# Autodesk Inventor assembly: Extended 5 frame Hole Top and Bottom
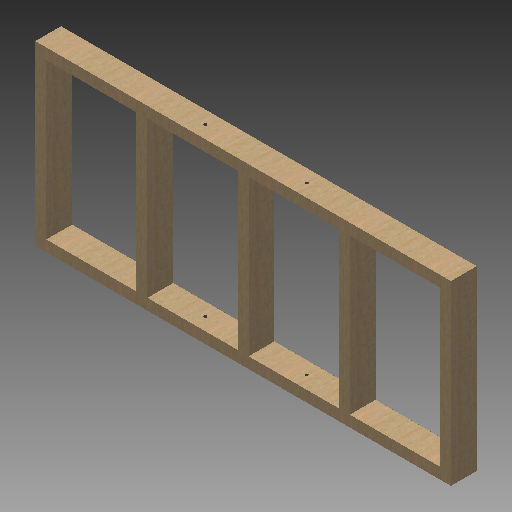
[picture p0: Inventor's stored thumbnail of the model, 512x512]
Saved by Autodesk Inventor 2017 (Build 210142000, 142)
## iProperties
Created: 2017-05-26
Part Number: Extended 5 frame Hole Top and Bottom
Document SubType Name: Assembly
Designer: cas7
Author: cas7
## Documents named in this file (3)
- C:\Users\mcgratta\Documents\FDS_Validation_Test_Reports\NIST_Vent_Study\Inventor_NIST_Vent_Study\Assemblies\Extended 5 frame Hole Top and Bottom.iam
- C:\Users\mcgratta\Documents\FDS_Validation_Test_Reports\NIST_Vent_Study\Inventor_NIST_Vent_Study\Parts\56.25in 2x4.ipt
- C:\Users\mcgratta\Documents\FDS_Validation_Test_Reports\NIST_Vent_Study\Inventor_NIST_Vent_Study\Parts\21in 2x4.ipt
## Components (7 placed, 2 different names)
1. 56.25in 2x4:1 — Mate:1, Mate:5, Mate:7, Mate:9, Mate:10, Mate:11, Mate:12, Mate:13, Mate:14
2. 56.25in 2x4:2 — Mate:2, Mate:3, Mate:4, Mate:6, Mate:8
3. 4ft 2x4:1 — Mate:9, Mate:10
4. 4ft 2x4:2 — Mate:11, Mate:12
5. 4ft 2x4:3 — Mate:6, Mate:7, Mate:8
6. 4ft 2x4:4 — Mate:13, Mate:14
7. 4ft 2x4:5 — Mate:1, Mate:2, Mate:3, Mate:4, Mate:5
## Relationships (14: Mate 14)
- Mate:1: 56.25in 2x4:1 ↔ 4ft 2x4:5
- Mate:2: 56.25in 2x4:2 ↔ 4ft 2x4:5
- Mate:3: 56.25in 2x4:2 ↔ 4ft 2x4:5
- Mate:4: 56.25in 2x4:2 ↔ 4ft 2x4:5
- Mate:5: 56.25in 2x4:1 ↔ 4ft 2x4:5
- Mate:6: 56.25in 2x4:2 ↔ 4ft 2x4:3
- Mate:7: 56.25in 2x4:1 ↔ 4ft 2x4:3
- Mate:8: 56.25in 2x4:2 ↔ 4ft 2x4:3
- Mate:9: 56.25in 2x4:1 ↔ 4ft 2x4:1
- Mate:10: 56.25in 2x4:1 ↔ 4ft 2x4:1
- Mate:11: 56.25in 2x4:1 ↔ 4ft 2x4:2
- Mate:12: 56.25in 2x4:1 ↔ 4ft 2x4:2
- Mate:13: 56.25in 2x4:1 ↔ 4ft 2x4:4
- Mate:14: 56.25in 2x4:1 ↔ 4ft 2x4:4
